# Autodesk Inventor assembly: MR-20CNB_MRS20-1200_0
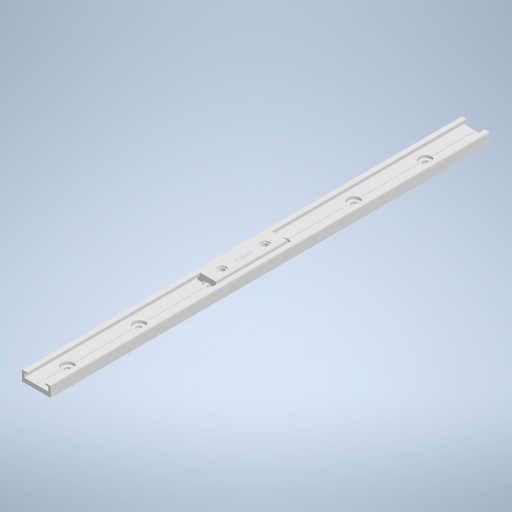
[picture p0: Inventor's stored thumbnail of the model, 512x512]
Saved by Autodesk Inventor 2023 (Build 270158000, 158)
## iProperties
Created: 2020-09-01
Part Number: MR-20CNB_MRS20-1200_0
Description: STEP AP203
Document SubType Name: Assembly
Designer: morita masato
Sending System: SolidWorks 2017
Preprocessor: SwSTEP 2.0
Title: MR-20CNB_MRS20-1200_0.step
Revision Number: ANY
## Documents named in this file (3)
- C:\Users\zegi\OneDrive - Kyushu University\2023NHK_RR_2ndvid\000_parts_zegi\slider\mr-20cnb_mrs20-1200_0.iam
- C:\Users\zegi\OneDrive - Kyushu University\2023NHK_RR_2ndvid\000_parts_zegi\slider\MR-20CNB.iam
- C:\Users\zegi\OneDrive - Kyushu University\2023NHK_RR_2ndvid\000_parts_zegi\slider\mrs20-1200.ipt
## Components (2 placed, 2 different names)
1. MR-20CNB_1 [sub-assembly] — メイト:1, メイト:2, メイト:3
2. mrs20-1200_2 — メイト:1, メイト:2, メイト:3
## Relationships (3: Mate 3)
- メイト:1 [Mate]: MR-20CNB_1 ↔ mrs20-1200_2
- メイト:2 [Mate] (0.1 mm): MR-20CNB_1 ↔ mrs20-1200_2
- メイト:3 [Mate] (0.1 mm): MR-20CNB_1 ↔ mrs20-1200_2
